# Autodesk Inventor assembly: SansCapacFata_Ricea f. Florentina alexandra-T7
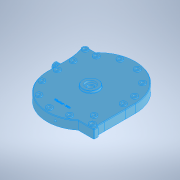
[picture p0: Inventor's stored thumbnail of the model, 180x180]
Saved by Autodesk Inventor 2022 (Build 260153000, 153)
## iProperties
Student_ACE: Ricea f. Florentina alexandra
Grupa_ACE: CR-3
Tema_ACE: 7-Ansamblu motor Wankel
An_ACE: 2022
Created: 2022-02-18
Part Number: SansCapacFata_Ricea f. Florentina alexandra-T7
Document SubType Name: Assembly
Designer: mtrot
Author: mtrot
## Documents named in this file (4)
- C:\1.GAC\tema7_var2\SansCapacFata_Ricea f. Florentina alexandra-T7.iam
- C:\1.GAC\tema7_var2\CapacFata.ipt
- C:\1.GAC\tema7_var2\Pinion.ipt
- C:\1.GAC\tema7_var2\SubansM4x10.iam
## Components (3 placed, 3 different names)
1. CapacFata:1 — Mate:1, Mate:2, Angle:1
2. Pinion:1 — Mate:1, Mate:2, Angle:1
3. SubansM4x10:1 [sub-assembly]
## Relationships (4: Mate 2, Angle 1, Insert 1)
- Mate:1: CapacFata:1 ↔ Pinion:1
- Mate:2: CapacFata:1 ↔ Pinion:1
- Angle:1 (99 deg): CapacFata:1 ↔ Pinion:1
- [Insert]: Pinion:1 ↔ SubansM4x10:1
